# Autodesk Inventor assembly: platform
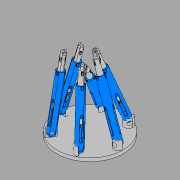
[picture p0: Inventor's stored thumbnail of the model, 180x180]
Saved by Autodesk Inventor 2020 (Build 240168000, 168)
## iProperties
Created: 2020-12-28
Part Number: platform
Document SubType Name: Assembly
Designer: freyja
Author: freyja
## Documents named in this file (3)
- C:\Users\freyja\Documents\OpenSpace\CAD\platform.iam
- C:\Users\freyja\Documents\OpenSpace\CAD\leg.iam
- C:\Users\freyja\Documents\OpenSpace\CAD\base.ipt
## Components (7 placed, 2 different names)
1. leg:1 [sub-assembly] — Mate:4, Mate:8
2. leg:2 [sub-assembly] — Mate:6, Mate:10
3. leg:3 [sub-assembly] — Mate:1, Mate:9
4. leg:4 [sub-assembly] — Mate:2, Mate:12
5. leg:5 [sub-assembly] — Mate:5, Mate:7
6. leg:6 [sub-assembly] — Mate:3, Mate:11
7. base:1 — Mate:1, Mate:2, Mate:3, Mate:4, Mate:5, Mate:6, Mate:7, Mate:8, Mate:9, Mate:10, Mate:11, Mate:12
## Relationships (12: Mate 12)
- Mate:1: leg:3 ↔ base:1
- Mate:2: leg:4 ↔ base:1
- Mate:3: leg:6 ↔ base:1
- Mate:4: leg:1 ↔ base:1
- Mate:5: leg:5 ↔ base:1
- Mate:6: leg:2 ↔ base:1
- Mate:7: leg:5 ↔ base:1
- Mate:8: leg:1 ↔ base:1
- Mate:9: leg:3 ↔ base:1
- Mate:10: leg:2 ↔ base:1
- Mate:11: leg:6 ↔ base:1
- Mate:12: leg:4 ↔ base:1
